# Autodesk Inventor assembly: y_holder
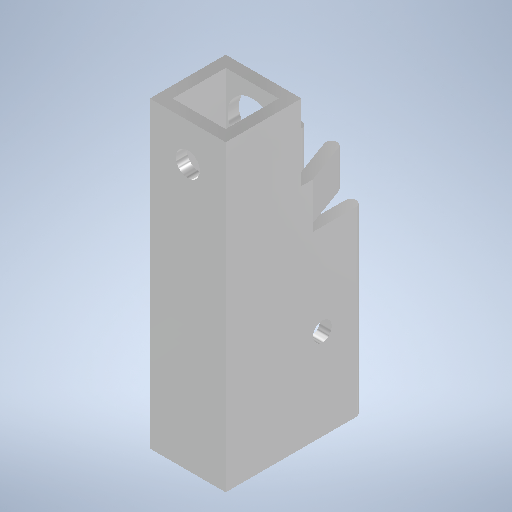
[picture p0: Inventor's stored thumbnail of the model, 512x512]
Saved by Autodesk Inventor 2025 (Build 290162000, 162)
## iProperties
Created: 2024-04-25
Part Number: y_holder
Document SubType Name: Assembly
Designer: KUPEC
Author: rader
## Documents named in this file (3)
- C:\Users\rader\Documents\rp\y_holder.iam
- C:\Users\rader\Documents\rp\y_holder.ipt
- C:\Users\rader\Documents\rp\y_standoff.ipt
## Components (2 placed, 2 different names)
1. y_holder:1 — Proti sobě:1, Vložit:1, Vložit:2
2. y_standoff:1 — Proti sobě:1, Vložit:1, Vložit:2
## Relationships (3: Insert 2, Mate 1)
- Proti sobě:1 [Mate]: y_holder:1 ↔ y_standoff:1
- Vložit:1 [Insert]: y_holder:1 ↔ y_standoff:1
- Vložit:2 [Insert]: y_holder:1 ↔ y_standoff:1
